# Autodesk Inventor assembly: CONTROLBOARDAS
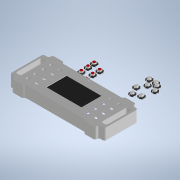
[picture p0: Inventor's stored thumbnail of the model, 180x180]
Saved by Autodesk Inventor 2020 (Build 240168000, 168)
## iProperties
Created: 2020-06-05
Part Number: CONTROLBOARDAS
Document SubType Name: Assembly
Designer: Gebruiker
Author: Gebruiker
## Documents named in this file (5)
- C:\Users\Gebruiker\Documents\GitHub\BeerMinder\3D-model\ControlBox\CONTROLBOARDAS.iam
- C:\Users\Gebruiker\Documents\GitHub\BeerMinder\3D-model\ControlBox\CONTROL_BOARD.ipt
- C:\Users\Gebruiker\Documents\GitHub\BeerMinder\3D-model\ControlBox\Nextion 4.3 Enhanced v10.ipt
- C:\Users\Gebruiker\Documents\GitHub\BeerMinder\3D-model\ControlBox\Tactal Switch - THRU(12mmx12mm - Illuminated - Red.ipt
- C:\Users\Gebruiker\Documents\GitHub\BeerMinder\3D-model\ControlBox\Tactal Switch - THRU(12mmx12mm - Illuminated - White.ipt
## Components (17 placed, 4 different names)
1. CONTROL_BOARD:1 — Mate:1, Angle:1, Angle:2, Mate:2
2. Nextion 4.3 Enhanced v10:1 — Mate:1, Angle:1, Angle:2, Mate:2
3. Tactal Switch - THRU(12mmx12mm - Illuminated - Red:1
4. Tactal Switch - THRU(12mmx12mm - Illuminated - Red:2
5. Tactal Switch - THRU(12mmx12mm - Illuminated - Red:3
6. Tactal Switch - THRU(12mmx12mm - Illuminated - Red:4
7. Tactal Switch - THRU(12mmx12mm - Illuminated - Red:5
8. Tactal Switch - THRU(12mmx12mm - Illuminated - Red:6
9. Tactal Switch - THRU(12mmx12mm - Illuminated - Red:7
10. Tactal Switch - THRU(12mmx12mm - Illuminated - White:1
11. Tactal Switch - THRU(12mmx12mm - Illuminated - White:2
12. Tactal Switch - THRU(12mmx12mm - Illuminated - White:3
13. Tactal Switch - THRU(12mmx12mm - Illuminated - White:4
14. Tactal Switch - THRU(12mmx12mm - Illuminated - White:5
15. Tactal Switch - THRU(12mmx12mm - Illuminated - White:6
16. Tactal Switch - THRU(12mmx12mm - Illuminated - White:7
17. Tactal Switch - THRU(12mmx12mm - Illuminated - White:8
## Relationships (4: Mate 2, Angle 2)
- Mate:1: CONTROL_BOARD:1 ↔ Nextion 4.3 Enhanced v10:1
- Angle:1 (0 deg): CONTROL_BOARD:1 ↔ Nextion 4.3 Enhanced v10:1
- Angle:2 (0 deg): CONTROL_BOARD:1 ↔ Nextion 4.3 Enhanced v10:1
- Mate:2: CONTROL_BOARD:1 ↔ Nextion 4.3 Enhanced v10:1
